# Autodesk Inventor assembly: Gears
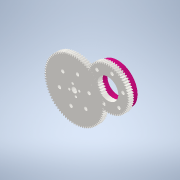
[picture p0: Inventor's stored thumbnail of the model, 180x180]
Saved by Autodesk Inventor 2020 (Build 240168000, 168)
## iProperties
Created: 2023-01-07
Part Number: Gears
Document SubType Name: Assembly
Designer: Allan
Author: Allan
## Documents named in this file (4)
- C:\Users\Jason\Documents\Inventor\FTC Robot 2023\Gears.iam
- C:\Users\Jason\Documents\Inventor\FTC Robot 2023\FTC Wheel Motor Gear.ipt
- C:\Users\Jason\Documents\Inventor\FTC Robot 2023\FTC Wheel Gear.ipt
- C:\Users\Jason\Documents\Inventor\FTC Robot 2023\Gears\Design Accelerator\Spur Gears1.iam
## Components (3 placed, 3 different names)
1. FTC Wheel Motor Gear:1 — Mate:1, Mate:2
2. FTC Wheel Gear:1 — Mate:3, Mate:4
3. Spur Gears:1 [sub-assembly] — Mate:1, Mate:2, Mate:3, Mate:4
## Relationships (4: Mate 4)
- Mate:1: FTC Wheel Motor Gear:1 ↔ Spur Gears:1
- Mate:2: FTC Wheel Motor Gear:1 ↔ Spur Gears:1
- Mate:3: FTC Wheel Gear:1 ↔ Spur Gears:1
- Mate:4: FTC Wheel Gear:1 ↔ Spur Gears:1
